# Autodesk Inventor assembly: Existing_Kitchen_And_Dining_Room
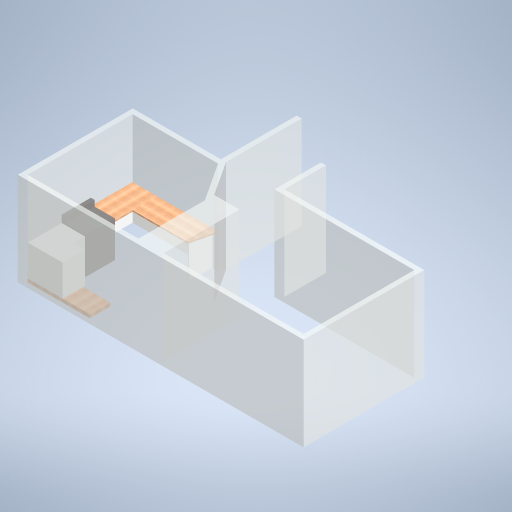
[picture p0: Inventor's stored thumbnail of the model, 512x512]
Saved by Autodesk Inventor 2024 (Build 280153000, 153)
## iProperties
Created: 2023-05-06
Part Number: Existing_Kitchen_And_Dining_Room
Document SubType Name: Assembly
Designer: Tom
Author: Tom
## Documents named in this file (6)
- C:\Users\Tom\Documents\Tom_Levers_Public_Git_Repository\Inventor\Mobility\Existing_Kitchen_And_Dining_Room.iam
- C:\Users\Tom\Documents\Tom_Levers_Public_Git_Repository\Inventor\Mobility\Walls--Existing_Kitchen_And_Dining_Room.ipt
- C:\Users\Tom\Documents\Tom_Levers_Public_Git_Repository\Inventor\Mobility\Stand--Sink_and_Corner_Cabinets.ipt
- C:\Users\Tom\Documents\Tom_Levers_Public_Git_Repository\Inventor\Mobility\Corner_Cabinet.ipt
- C:\Users\Tom\Documents\Tom_Levers_Public_Git_Repository\Inventor\Mobility\Range.ipt
- C:\Users\Tom\Documents\Tom_Levers_Public_Git_Repository\Inventor\Mobility\Window_Cabinet\Window_Cabinet.iam
## Components (5 placed, 5 different names)
1. Walls--Existing_Kitchen_And_Dining_Room:1 — Mate:1, Mate:2, Flush:1, Mate:3, Mate:4, Mate:6, Flush:2, Mate:8, Mate:9, Flush:3
2. Stand--Sink_and_Corner_Cabinets:1 — Mate:1, Mate:2, Flush:1, Mate:5
3. Corner_Cabinet:1 — Mate:3, Mate:4, Mate:5, Mate:7
4. Range:1 — Mate:6, Mate:7, Flush:2
5. Window_Cabinet:1 [sub-assembly] — Mate:8, Mate:9, Flush:3
## Relationships (12: Mate 9, Flush 3)
- Mate:1: Walls--Existing_Kitchen_And_Dining_Room:1 ↔ Stand--Sink_and_Corner_Cabinets:1
- Mate:2: Walls--Existing_Kitchen_And_Dining_Room:1 ↔ Stand--Sink_and_Corner_Cabinets:1
- Flush:1: Walls--Existing_Kitchen_And_Dining_Room:1 ↔ Stand--Sink_and_Corner_Cabinets:1
- Mate:3: Walls--Existing_Kitchen_And_Dining_Room:1 ↔ Corner_Cabinet:1
- Mate:4: Walls--Existing_Kitchen_And_Dining_Room:1 ↔ Corner_Cabinet:1
- Mate:5: Stand--Sink_and_Corner_Cabinets:1 ↔ Corner_Cabinet:1
- Mate:6: Walls--Existing_Kitchen_And_Dining_Room:1 ↔ Range:1
- Mate:7: Corner_Cabinet:1 ↔ Range:1
- Flush:2: Walls--Existing_Kitchen_And_Dining_Room:1 ↔ Range:1
- Mate:8: Walls--Existing_Kitchen_And_Dining_Room:1 ↔ Window_Cabinet:1
- Mate:9: Walls--Existing_Kitchen_And_Dining_Room:1 ↔ Window_Cabinet:1
- Flush:3: Walls--Existing_Kitchen_And_Dining_Room:1 ↔ Window_Cabinet:1
